# Autodesk Inventor assembly: Parallax_Ping_Sensor
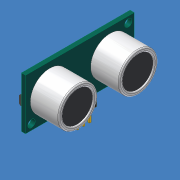
[picture p0: Inventor's stored thumbnail of the model, 180x180]
Saved by Autodesk Inventor 2012 (Build 160160000, 160)
## iProperties
Category: FIRST
Manager: Ed Sparks
Company: FirstCadLibrary
Shininess: 64.0
Length Units: 11272
Angle Units: 11279
Time Units: 11290
Mass Units: 11286
Length Display Precision: 3
Angle Display Precision: 2
Compacted: True
Part Number: Parallax_Ping_Sensor
Document SubType Name: Assembly
Created: 2007-12-18
Designer: Owner
Project: FIRST
Catalog Web Link: www.firstcadlibrary.com
Engineer: Ed Sparks
Mass: 7.86138 g
Surface Area: 50.1079 cm^2
Volume: 6.83497 cm^3
Density: 1.15017 g/cm^3
Density: 0.0
Volumn: 0.0
Area: 0.0
PropertySet Name: Model Information
Control State: 0
Master: False
Checked Out: False
Author: Owner
Keywords: FIRST
## Documents named in this file (6)
- C:\Users\Admin\Documents\Inventor\SumoJaime2012\Parallax Ping Sensor.iam
- C:\Users\Admin\Documents\Inventor\SumoJaime2012\Parallax Ping PCB.ipt
- C:\Users\Admin\Documents\Inventor\SumoJaime2012\Parallax Ping Transducer.ipt
- C:\Users\Admin\Documents\Inventor\SumoJaime2012\Cap1 SMT.ipt
- C:\Users\Admin\Documents\Inventor\SumoJaime2012\14 Pin SMT.ipt
- C:\Users\Admin\Documents\Inventor\SumoJaime2012\3 Pin Header 90 Degree.ipt
## Components (13 placed, 5 different names)
1. Parallax Ping PCB:1 — Mate:1, Mate:2, Mate:3, Mate:4, Mate:5, Mate:6, Mate:7, Flush:1, Flush:2, Mate:8, Flush:3, Flush:4, Mate:9, Mate:10, Flush:5, Mate:11, Flush:6, Flush:7
2. Parallax Ping Transducer:1 — Mate:2, Mate:3, Mate:5
3. Parallax Ping Transducer:2 — Mate:1, Mate:4, Mate:6
4. 3 Pin Header 90 Degree:1 — Mate:11, Flush:6, Flush:7
5. Cap1 SMT:1 — Mate:7, Flush:1, Flush:2
6. Cap1 SMT:2
7. Cap1 SMT:3
8. Cap1 SMT:4 — Mate:8, Flush:3, Flush:4
9. Cap1 SMT:5
10. Cap1 SMT:6
11. 14 Pin SMT:1 — Mate:9, Mate:10, Flush:5
12. 14 Pin SMT:2
13. 14 Pin SMT:3
## Component patterns: (3 elements, first: Cap1 SMT:1), (3 elements, first: Cap1 SMT:4), (3 elements, first: 14 Pin SMT:1)
## Relationships (18: Mate 11, Flush 7)
- Mate:1: Parallax Ping PCB:1 ↔ Parallax Ping Transducer:2
- Mate:2: Parallax Ping PCB:1 ↔ Parallax Ping Transducer:1
- Mate:3 (10.668 mm): Parallax Ping PCB:1 ↔ Parallax Ping Transducer:1
- Mate:4 (10.668 mm): Parallax Ping PCB:1 ↔ Parallax Ping Transducer:2
- Mate:5 (10.16 mm): Parallax Ping PCB:1 ↔ Parallax Ping Transducer:1
- Mate:6 (10.16 mm): Parallax Ping PCB:1 ↔ Parallax Ping Transducer:2
- Mate:7: Parallax Ping PCB:1 ↔ Cap1 SMT:1
- Flush:1 (13.208 mm): Parallax Ping PCB:1 ↔ Cap1 SMT:1
- Flush:2 (-2.54 mm): Parallax Ping PCB:1 ↔ Cap1 SMT:1
- Mate:8: Parallax Ping PCB:1 ↔ Cap1 SMT:4
- Flush:3 (2.54 mm): Parallax Ping PCB:1 ↔ Cap1 SMT:4
- Flush:4 (13.208 mm): Parallax Ping PCB:1 ↔ Cap1 SMT:4
- Mate:9: Parallax Ping PCB:1 ↔ 14 Pin SMT:1
- Mate:10: Parallax Ping PCB:1 ↔ 14 Pin SMT:1
- Flush:5 (0.508 mm): Parallax Ping PCB:1 ↔ 14 Pin SMT:1
- Mate:11: Parallax Ping PCB:1 ↔ 3 Pin Header 90 Degree:1
- Flush:6: Parallax Ping PCB:1 ↔ 3 Pin Header 90 Degree:1
- Flush:7 (-2 mm): Parallax Ping PCB:1 ↔ 3 Pin Header 90 Degree:1
